# Autodesk Inventor assembly: Sport57 with Redline and 4inc wheel
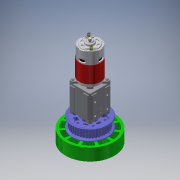
[picture p0: Inventor's stored thumbnail of the model, 180x180]
Saved by Autodesk Inventor 2018 (Build 220112000, 112)
## iProperties
Created: 2018-01-18
Part Number: Sport57 with Redline and 4inc wheel
Document SubType Name: Assembly
Designer: Apple
Author: Apple
## Documents named in this file (5)
- C:\Users\Apple\Documents\Inventor\2018 PowerUp\Cube Intake\Sport57 with Redline and 4inc wheel.iam
- C:\Users\Apple\Documents\Inventor\2018 PowerUp\AndyMark\am-3755+-+20_1+-+57+Sport.ipt
- C:\Users\Apple\Documents\Inventor\2018 PowerUp\AndyMark\am-3775+RedLine+Motor.ipt
- C:\Users\Apple\Documents\Inventor\2018 PowerUp\AndyMark\am-3480+4IN+500Hex+Bore+Compliant+Wheel.ipt
- C:\Users\Apple\Documents\Inventor\2018 PowerUp\AndyMark\42toothHTDpulleyHalfRev2.ipt
## Components (5 placed, 4 different names)
1. am-3755+-+20_1+-+57+Sport:1 — Mate:1, Mate:2, Mate:3, Mate:9
2. am-3775+RedLine+Motor:1 — Mate:1, Mate:2
3. am-3480+4IN+500Hex+Bore+Compliant+Wheel:1 — Mate:3, Mate:7, Mate:8
4. 42toothHTDpulleyHalfRev2:1 — Mate:4, Mate:5, Mate:6, Mate:8
5. 42toothHTDpulleyHalfRev2:2 — Mate:4, Mate:5, Mate:6, Mate:7, Mate:9
## Relationships (9: Mate 9)
- Mate:1: am-3755+-+20_1+-+57+Sport:1 ↔ am-3775+RedLine+Motor:1
- Mate:2: am-3755+-+20_1+-+57+Sport:1 ↔ am-3775+RedLine+Motor:1
- Mate:3: am-3755+-+20_1+-+57+Sport:1 ↔ am-3480+4IN+500Hex+Bore+Compliant+Wheel:1
- Mate:4: 42toothHTDpulleyHalfRev2:1 ↔ 42toothHTDpulleyHalfRev2:2
- Mate:5: 42toothHTDpulleyHalfRev2:1 ↔ 42toothHTDpulleyHalfRev2:2
- Mate:6: 42toothHTDpulleyHalfRev2:1 ↔ 42toothHTDpulleyHalfRev2:2
- Mate:7: am-3480+4IN+500Hex+Bore+Compliant+Wheel:1 ↔ 42toothHTDpulleyHalfRev2:2
- Mate:8 (-25.4 mm): am-3480+4IN+500Hex+Bore+Compliant+Wheel:1 ↔ 42toothHTDpulleyHalfRev2:1
- Mate:9 (3.175 mm): am-3755+-+20_1+-+57+Sport:1 ↔ 42toothHTDpulleyHalfRev2:2
